# Autodesk Inventor assembly: CubeAssembly
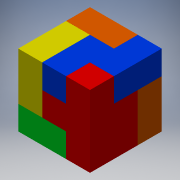
[picture p0: Inventor's stored thumbnail of the model, 180x180]
Saved by Autodesk Inventor 2019 (Build 230136000, 136)
## iProperties
Created: 2019-09-11
Part Number: CubeAssembly
Document SubType Name: Assembly
Designer: IED8
Author: IED8
## Documents named in this file (6)
- C:\Users\IED8\Documents\Giovanni's InvDes\Projects\CubePuzzleDesigns\CubeAssembly.iam
- C:\Users\IED8\Documents\Giovanni's InvDes\Projects\CubePuzzleDesigns\CubePart1.ipt
- C:\Users\IED8\Documents\Giovanni's InvDes\Projects\CubePuzzleDesigns\CubePart2.ipt
- C:\Users\IED8\Documents\Giovanni's InvDes\Projects\CubePuzzleDesigns\CubePart3.ipt
- C:\Users\IED8\Documents\Giovanni's InvDes\Projects\CubePuzzleDesigns\CubePart5.ipt
- C:\Users\IED8\Documents\Giovanni's InvDes\Projects\CubePuzzleDesigns\CubePart4.ipt
## Components (5 placed, 5 different names)
1. CubePart1:1 — Mate:1, Flush:1, Flush:2, Flush:4, Mate:2, Flush:5, Flush:7
2. CubePart2:1 — Mate:1, Flush:1, Flush:2, Flush:3, Flush:9
3. CubePart3:1 — Flush:3, Flush:4, Mate:2, Flush:5, Flush:6, Mate:3, Mate:4, Flush:8
4. CubePart5:1 — Flush:6, Mate:3, Mate:4
5. CubePart4:1 — Flush:7, Flush:8, Flush:9
## Relationships (13: Flush 9, Mate 4)
- Mate:1: CubePart1:1 ↔ CubePart2:1
- Flush:1: CubePart1:1 ↔ CubePart2:1
- Flush:2: CubePart1:1 ↔ CubePart2:1
- Flush:3: CubePart2:1 ↔ CubePart3:1
- Flush:4: CubePart1:1 ↔ CubePart3:1
- Mate:2: CubePart1:1 ↔ CubePart3:1
- Flush:5: CubePart1:1 ↔ CubePart3:1
- Flush:6: CubePart3:1 ↔ CubePart5:1
- Mate:3: CubePart3:1 ↔ CubePart5:1
- Mate:4: CubePart3:1 ↔ CubePart5:1
- Flush:7: CubePart1:1 ↔ CubePart4:1
- Flush:8: CubePart3:1 ↔ CubePart4:1
- Flush:9: CubePart2:1 ↔ CubePart4:1
